# Autodesk Inventor assembly: enc-TopPanel - Assembly no Absorber
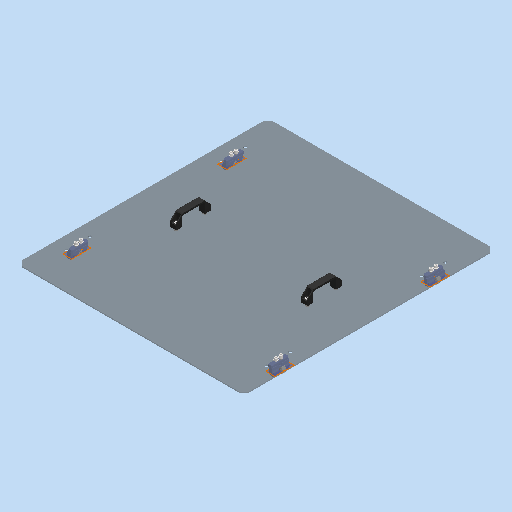
[picture p0: Inventor's stored thumbnail of the model, 512x512]
Saved by Autodesk Inventor 2023.2 (Build 272271000, 271)
## iProperties
Created: 2023-11-30
Part Number: enc-TopPanel - Assembly no Absorber
Document SubType Name: Assembly
Designer: Nils Bade
Author: Nils Bade
## Documents named in this file (6)
- C:\Users\nilsb\Documents\Inventor\Projektarbeit-Bade\Enclosure\enc-TopPanel - Assembly no Absorber.iam
- C:\Users\nilsb\Documents\Inventor\Projektarbeit-Bade\Enclosure\enc-TopPanel.ipt
- C:\Users\nilsb\Documents\Inventor\Projektarbeit-Bade\Enclosure\V-Slot Door Handle v1.ipt
- C:\Users\nilsb\Documents\Inventor\Projektarbeit-Bade\Schrauben\Cap Head Screw M6x16 - DIN912.ipt
- C:\Users\nilsb\Documents\Inventor\Projektarbeit-Bade\RatRig_Standards\Hex Locking Nut - M6 v2.ipt
- C:\Users\nilsb\Documents\Inventor\Projektarbeit-Bade\Enclosure\Magnet PanelFrame 90deg connected.iam
## Components (15 placed, 5 different names)
1. enc-TopPanel:1 — Passend:1, Passend:2, Passend:3, Passend:4, Passend:5, Passend:6, Passend:19, Passend:20, Passend:21, Passend:22, Passend:35, Passend:36, Passend:37, Passend:38
2. V-Slot Door Handle v1:1 — Passend:3, Passend:4, Passend:5, Passend:9, Passend:10, Passend:11, Passend:12
3. V-Slot Door Handle v1:2 — Passend:1, Passend:2, Passend:6, Passend:7, Passend:8, Passend:13, Passend:14
4. Cap Head Screw M6x16 - DIN912:1 — Passend:7, Passend:13, Passend:17
5. Cap Head Screw M6x16 - DIN912:2 — Passend:8, Passend:14, Passend:18
6. Cap Head Screw M6x16 - DIN912:3 — Passend:9, Passend:11, Passend:16
7. Cap Head Screw M6x16 - DIN912:4 — Passend:10, Passend:12, Passend:15
8. Hex Locking Nut - M6 v2:1 — Passend:18, Passend:20
9. Hex Locking Nut - M6 v2:2 — Passend:17, Passend:19
10. Hex Locking Nut - M6 v2:3 — Passend:16, Passend:22
11. Hex Locking Nut - M6 v2:4 — Passend:15, Passend:21
12. Magnet PanelFrame 90deg connected:3 [sub-assembly]
13. Magnet PanelFrame 90deg connected:4 [sub-assembly]
14. Magnet PanelFrame 90deg connected:2 [sub-assembly] — Passend:35, Passend:36
15. Magnet PanelFrame 90deg connected:1 [sub-assembly] — Passend:37, Passend:38
## Relationships (34: Mate 34)
- Passend:1 [Mate]: enc-TopPanel:1 ↔ V-Slot Door Handle v1:2
- Passend:2 [Mate]: enc-TopPanel:1 ↔ V-Slot Door Handle v1:2
- Passend:3 [Mate]: enc-TopPanel:1 ↔ V-Slot Door Handle v1:1
- Passend:4 [Mate]: enc-TopPanel:1 ↔ V-Slot Door Handle v1:1
- Passend:5 [Mate]: enc-TopPanel:1 ↔ V-Slot Door Handle v1:1
- Passend:6 [Mate]: enc-TopPanel:1 ↔ V-Slot Door Handle v1:2
- Passend:7 [Mate]: V-Slot Door Handle v1:2 ↔ Cap Head Screw M6x16 - DIN912:1
- Passend:8 [Mate]: V-Slot Door Handle v1:2 ↔ Cap Head Screw M6x16 - DIN912:2
- Passend:9 [Mate]: V-Slot Door Handle v1:1 ↔ Cap Head Screw M6x16 - DIN912:3
- Passend:10 [Mate]: V-Slot Door Handle v1:1 ↔ Cap Head Screw M6x16 - DIN912:4
- Passend:11 [Mate]: V-Slot Door Handle v1:1 ↔ Cap Head Screw M6x16 - DIN912:3
- Passend:12 [Mate]: V-Slot Door Handle v1:1 ↔ Cap Head Screw M6x16 - DIN912:4
- Passend:13 [Mate]: V-Slot Door Handle v1:2 ↔ Cap Head Screw M6x16 - DIN912:1
- Passend:14 [Mate]: V-Slot Door Handle v1:2 ↔ Cap Head Screw M6x16 - DIN912:2
- Passend:15 [Mate]: Cap Head Screw M6x16 - DIN912:4 ↔ Hex Locking Nut - M6 v2:4
- Passend:16 [Mate]: Cap Head Screw M6x16 - DIN912:3 ↔ Hex Locking Nut - M6 v2:3
- Passend:17 [Mate]: Cap Head Screw M6x16 - DIN912:1 ↔ Hex Locking Nut - M6 v2:2
- Passend:18 [Mate]: Cap Head Screw M6x16 - DIN912:2 ↔ Hex Locking Nut - M6 v2:1
- Passend:19 [Mate]: enc-TopPanel:1 ↔ Hex Locking Nut - M6 v2:2
- Passend:20 [Mate]: enc-TopPanel:1 ↔ Hex Locking Nut - M6 v2:1
- Passend:21 [Mate]: enc-TopPanel:1 ↔ Hex Locking Nut - M6 v2:4
- Passend:22 [Mate]: enc-TopPanel:1 ↔ Hex Locking Nut - M6 v2:3
- [Mate]: enc-TopPanel:1 ↔ Magnet PanelFrame 90deg connected:3
- [Mate]: enc-TopPanel:1 ↔ Magnet PanelFrame 90deg connected:3
- [Mate]: enc-TopPanel:1 ↔ Magnet PanelFrame 90deg connected:3
- [Mate]: enc-TopPanel:1 ↔ Magnet PanelFrame 90deg connected:4
- [Mate]: enc-TopPanel:1 ↔ Magnet PanelFrame 90deg connected:4
- [Mate]: enc-TopPanel:1 ↔ Magnet PanelFrame 90deg connected:4
- [Mate]: enc-TopPanel:1 ↔ Magnet PanelFrame 90deg connected:1
- [Mate]: enc-TopPanel:1 ↔ Magnet PanelFrame 90deg connected:2
- Passend:35 [Mate]: enc-TopPanel:1 ↔ Magnet PanelFrame 90deg connected:2
- Passend:36 [Mate]: enc-TopPanel:1 ↔ Magnet PanelFrame 90deg connected:2
- Passend:37 [Mate]: enc-TopPanel:1 ↔ Magnet PanelFrame 90deg connected:1
- Passend:38 [Mate]: enc-TopPanel:1 ↔ Magnet PanelFrame 90deg connected:1
